# Autodesk Inventor assembly: MainPhalangeAssembly
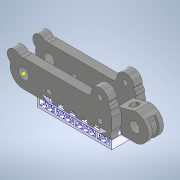
[picture p0: Inventor's stored thumbnail of the model, 180x180]
Saved by Autodesk Inventor 2020 (Build 240168000, 168)
## iProperties
Created: 2020-05-08
Part Number: MainPhalangeAssembly
Document SubType Name: Assembly
Designer: Ajay Yadiki
Author: Ajay Yadiki
## Documents named in this file (4)
- C:\Users\Ajay Yadiki\Desktop\Project Gripper\MainPhalangeAssembly.iam
- C:\Users\Ajay Yadiki\Desktop\Project Gripper\MainPhalange.ipt
- C:\Users\Ajay Yadiki\Desktop\Project Gripper\MainPhalange_grip_support.ipt
- C:\Users\Ajay Yadiki\Desktop\Project Gripper\MainPhalange_grip.ipt
## Components (3 placed, 3 different names)
1. MainPhalange:1 — Mate:1, Flush:1, Mate:2, Flush:2, Flush:3, Mate:3
2. MainPhalange_grip_support:1 — Mate:1, Flush:1, Mate:2
3. MainPhalange_grip:1 — Flush:2, Flush:3, Mate:3
## Relationships (6: Mate 3, Flush 3)
- Mate:1: MainPhalange:1 ↔ MainPhalange_grip_support:1
- Flush:1: MainPhalange:1 ↔ MainPhalange_grip_support:1
- Mate:2 (0.254 mm): MainPhalange:1 ↔ MainPhalange_grip_support:1
- Flush:2: MainPhalange:1 ↔ MainPhalange_grip:1
- Flush:3: MainPhalange:1 ↔ MainPhalange_grip:1
- Mate:3: MainPhalange:1 ↔ MainPhalange_grip:1
